# Autodesk Inventor assembly: main_sumec_assembly
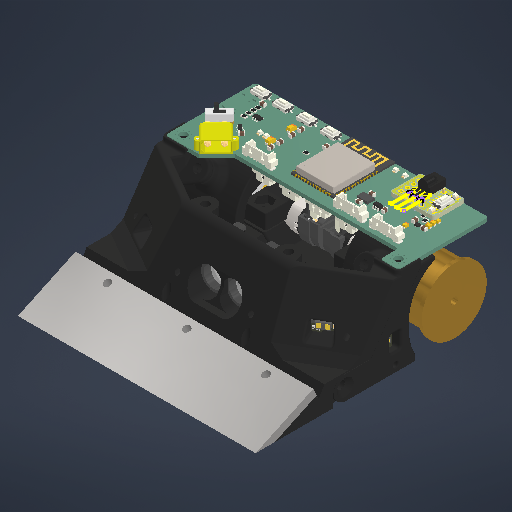
[picture p0: Inventor's stored thumbnail of the model, 512x512]
Saved by Autodesk Inventor 2025 (Build 290162000, 162)
## iProperties
Created: 2025-03-23
Part Number: main_sumec_assembly
Document SubType Name: Assembly
Designer: Simak
Author: Simak
## Documents named in this file (13)
- C:\GitHub\Sumec-MiniSumo-MECH\main_sumec_assembly.iam
- C:\GitHub\Sumec-MiniSumo-MECH\3D_printed\body-main.ipt
- C:\GitHub\Sumec-MiniSumo-MECH\3D_printed\body-front.ipt
- C:\GitHub\Sumec-MiniSumo-MECH\3D_printed\body-motor_comparment.ipt
- C:\GitHub\Sumec-MiniSumo-MECH\3D_printed\motor_C_clamp.ipt
- C:\GitHub\Sumec-MiniSumo-MECH\electronics\AssemBeneWake TF-LUNA.ipt
- C:\GitHub\Sumec-MiniSumo-MECH\electronics\pololu_12v_650rpm-cb-enc-side-con.ipt
- C:\GitHub\Sumec-MiniSumo-MECH\electronics\pololu-digital-distance-sensor-irs17a.ipt
- C:\GitHub\Sumec-MiniSumo-MECH\electronics\PCBs\main board\SUMEC_MK_V .iam
- C:\GitHub\Sumec-MiniSumo-MECH\machined\JSUMO_Wheel_33x25mm.ipt
- C:\GitHub\Sumec-MiniSumo-MECH\machined\lowerRamp.ipt
- C:\GitHub\Sumec-MiniSumo-MECH\odher\qreMiniBoard2.ipt
- C:\GitHub\Sumec-MiniSumo-MECH\machined\wheelGen2.ipt
## Components (17 placed, 12 different names)
1. body-main:1 — Vložit:1, openLock, Vložit:2, Úhel:1, Vložit:5, Stejný směr:4, Vložit:6, Stejný směr:5, Stejný směr:8, Stejný směr:10, Stejný směr:12
2. body-front:1 — Vložit:1, openLock, Proti sobě:6, Stejný směr:3, Vložit:3, Vložit:4, Proti sobě:7, Vložit:7, Proti sobě:8, Vložit:8, Vložit:9, Vložit:10, Vložit:11, Stejný směr:11
3. body-motor_comparment:1 — Vložit:2, Úhel:1, Proti sobě:1, Proti sobě:2, Proti sobě:3, Proti sobě:4, Proti sobě:5, Stejný směr:2, Proti sobě:9, Stejný směr:6, Proti sobě:10, Proti sobě:11, Stejný směr:7, Proti sobě:12
4. motor_C_clamp:1 — Proti sobě:9, Stejný směr:6, Proti sobě:10
5. AssemBeneWake TF-LUNA:1 — Proti sobě:6, Stejný směr:3, Vložit:3
6. pololu_12v_650rpm-cb-enc-side-con:1 — Proti sobě:1, Proti sobě:2, Proti sobě:3, Proti sobě:15
7. pololu-digital-distance-sensor-irs17a:1 — Vložit:4, Proti sobě:7
8. pololu_12v_650rpm-cb-enc-side-con:2 — Proti sobě:4, Proti sobě:5, Stejný směr:2, Proti sobě:14
9. pololu-digital-distance-sensor-irs17a:2 — Vložit:7, Proti sobě:8
10. pololu-digital-distance-sensor-irs17a:3 — Vložit:5, Stejný směr:4
11. pololu-digital-distance-sensor-irs17a:4 — Vložit:6, Stejný směr:5
12. motor_C_clamp:2 — Proti sobě:11, Stejný směr:7, Proti sobě:12
13. SUMEC_MK_V :1 [sub-assembly] — Vložit:8, Stejný směr:8
14. lowerRamp:1 — Vložit:9, Vložit:10
15. JSUMO_Wheel_33x25mm:2 — Proti sobě:14, Stejný směr:10
16. qreMiniBoard2:1 — Vložit:11, Stejný směr:11
17. wheelGen2:1 — Proti sobě:15, Stejný směr:12
## Relationships (37: Mate 14, Insert 11, Flush 11, Angle 1)
- Vložit:1 [Insert]: body-main:1 ↔ body-front:1
- openLock [Flush]: body-main:1 ↔ body-front:1
- Vložit:2 [Insert] (0.75 mm): body-main:1 ↔ body-motor_comparment:1
- Úhel:1 [Angle] (0 deg): body-main:1 ↔ body-motor_comparment:1
- Proti sobě:1 [Mate]: body-motor_comparment:1 ↔ pololu_12v_650rpm-cb-enc-side-con:1
- Proti sobě:2 [Mate]: body-motor_comparment:1 ↔ pololu_12v_650rpm-cb-enc-side-con:1
- Proti sobě:3 [Mate]: body-motor_comparment:1 ↔ pololu_12v_650rpm-cb-enc-side-con:1
- Proti sobě:4 [Mate]: body-motor_comparment:1 ↔ pololu_12v_650rpm-cb-enc-side-con:2
- Proti sobě:5 [Mate]: body-motor_comparment:1 ↔ pololu_12v_650rpm-cb-enc-side-con:2
- Stejný směr:2 [Flush]: body-motor_comparment:1 ↔ pololu_12v_650rpm-cb-enc-side-con:2
- Proti sobě:6 [Mate]: body-front:1 ↔ AssemBeneWake TF-LUNA:1
- Stejný směr:3 [Flush]: body-front:1 ↔ AssemBeneWake TF-LUNA:1
- Vložit:3 [Insert]: body-front:1 ↔ AssemBeneWake TF-LUNA:1
- Vložit:4 [Insert]: body-front:1 ↔ pololu-digital-distance-sensor-irs17a:1
- Proti sobě:7 [Mate]: body-front:1 ↔ pololu-digital-distance-sensor-irs17a:1
- Vložit:5 [Insert]: body-main:1 ↔ pololu-digital-distance-sensor-irs17a:3
- Stejný směr:4 [Flush]: body-main:1 ↔ pololu-digital-distance-sensor-irs17a:3
- Vložit:6 [Insert]: body-main:1 ↔ pololu-digital-distance-sensor-irs17a:4
- Stejný směr:5 [Flush]: body-main:1 ↔ pololu-digital-distance-sensor-irs17a:4
- Vložit:7 [Insert]: body-front:1 ↔ pololu-digital-distance-sensor-irs17a:2
- Proti sobě:8 [Mate]: body-front:1 ↔ pololu-digital-distance-sensor-irs17a:2
- Proti sobě:9 [Mate]: body-motor_comparment:1 ↔ motor_C_clamp:1
- Stejný směr:6 [Flush]: body-motor_comparment:1 ↔ motor_C_clamp:1
- Proti sobě:10 [Mate]: body-motor_comparment:1 ↔ motor_C_clamp:1
- Proti sobě:11 [Mate]: body-motor_comparment:1 ↔ motor_C_clamp:2
- Stejný směr:7 [Flush]: body-motor_comparment:1 ↔ motor_C_clamp:2
- Proti sobě:12 [Mate]: body-motor_comparment:1 ↔ motor_C_clamp:2
- Vložit:8 [Insert]: body-front:1 ↔ SUMEC_MK_V :1
- Stejný směr:8 [Flush]: body-main:1 ↔ SUMEC_MK_V :1
- Vložit:9 [Insert]: body-front:1 ↔ lowerRamp:1
- Vložit:10 [Insert]: body-front:1 ↔ lowerRamp:1
- Proti sobě:14 [Mate]: pololu_12v_650rpm-cb-enc-side-con:2 ↔ JSUMO_Wheel_33x25mm:2
- Stejný směr:10 [Flush]: body-main:1 ↔ JSUMO_Wheel_33x25mm:2
- Vložit:11 [Insert]: body-front:1 ↔ qreMiniBoard2:1
- Stejný směr:11 [Flush]: body-front:1 ↔ qreMiniBoard2:1
- Proti sobě:15 [Mate]: pololu_12v_650rpm-cb-enc-side-con:1 ↔ wheelGen2:1
- Stejný směr:12 [Flush]: body-main:1 ↔ wheelGen2:1
